# Autodesk Inventor assembly: ASY GBK 3330 central wall shield 9
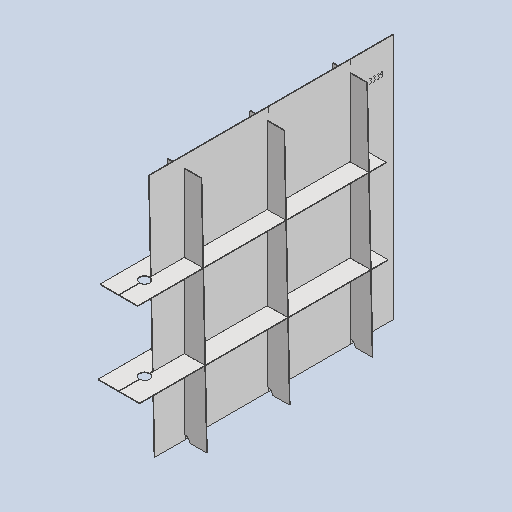
[picture p0: Inventor's stored thumbnail of the model, 512x512]
Saved by Autodesk Inventor 2026.3 (Build 303398000, 398)
## iProperties
Created: 2026-05-19
Part Number: ASY GBK 3330 central wall shield 9
Document SubType Name: Assembly
Designer: pokla
Mass: 123029 g
Surface Area: 79995.2 cm^2
Volume: 15672.5 cm^3
Density: 7.85 g/cm^3
Stock Number: 3330
Author: admin
## Documents named in this file (7)
- C:\Users\admin\Documents\Inventor\GBK-Gubkinskiy\ASY GBK 3330 central wall shield 9.iam
- C:\Users\admin\Documents\Inventor\GBK-Gubkinskiy\GBK 0101 main rib.ipt
- C:\Users\admin\Documents\Inventor\GBK-Gubkinskiy\GBK 3339 shield 9.ipt
- C:\Users\admin\Documents\Inventor\GBK-Gubkinskiy\GBK 3311 central third rib_CPY1.ipt
- GBK 3311 central third rib_CPY1.ipt
- C:\Users\admin\Documents\Inventor\GBK-Gubkinskiy\GBK 3312 stringer 7.ipt
- C:\Users\admin\Documents\Inventor\GBK-Gubkinskiy\GBK 3313 stringer 8.ipt
## Components (11 placed, 4 different names)
1. GBK 3312 stringer 7:1 — Rigid:1
2. GBK 3339 shield 9:1 — Mate:1, Mate:2, Mate:4, Flush:6, Mate:5, Flush:7, Flush:6
3. GBK 3313 stringer 8:1 — Rigid:2, Rigid:7, Rigid:8
4. GBK 3312 stringer 7:2 — Rigid:4
5. GBK 3313 stringer 8:2 — Rigid:3, Flush:6, Rigid:5, Rigid:6
6. GBK 3311 central third rib_CPY1:2 — Flush:4, Mate:5, Flush:7, Rigid:2, Rigid:1
7. GBK 3311 central third rib_CPY1:1 — Mate:4, Flush:6, Flush:4, Rigid:3, Rigid:4
8. GBK 3311 central third rib_CPY1:3 — Rigid:5
9. GBK 3311 central third rib_CPY1:4 — Rigid:6
10. GBK 3311 central third rib_CPY1:5 — Rigid:7
11. GBK 3311 central third rib_CPY1:6 — Rigid:8
## Relationships (16: WeldJoint 8, Mate 4, Flush 4)
- Mate:1: GBK 3339 shield 9:1
- Mate:2: GBK 3339 shield 9:1
- Mate:4: GBK 3339 shield 9:1 ↔ GBK 3311 central third rib_CPY1:1
- Flush:6: GBK 3339 shield 9:1 ↔ GBK 3311 central third rib_CPY1:1
- Flush:4: GBK 3311 central third rib_CPY1:2 ↔ GBK 3311 central third rib_CPY1:1
- Mate:5: GBK 3339 shield 9:1 ↔ GBK 3311 central third rib_CPY1:2
- Flush:7: GBK 3339 shield 9:1 ↔ GBK 3311 central third rib_CPY1:2
- Rigid:3 [WeldJoint] (4 mm): GBK 3313 stringer 8:2 ↔ GBK 3311 central third rib_CPY1:1
- Rigid:4 [WeldJoint] (4 mm): GBK 3312 stringer 7:2 ↔ GBK 3311 central third rib_CPY1:1
- Rigid:2 [WeldJoint] (4 mm): GBK 3313 stringer 8:1 ↔ GBK 3311 central third rib_CPY1:2
- Rigid:1 [WeldJoint] (4 mm): GBK 3312 stringer 7:1 ↔ GBK 3311 central third rib_CPY1:2
- Flush:6 (155 mm): GBK 3339 shield 9:1 ↔ GBK 3313 stringer 8:2
- Rigid:5 [WeldJoint] (4 mm): GBK 3313 stringer 8:2 ↔ GBK 3311 central third rib_CPY1:3
- Rigid:6 [WeldJoint] (4 mm): GBK 3313 stringer 8:2 ↔ GBK 3311 central third rib_CPY1:4
- Rigid:7 [WeldJoint] (4 mm): GBK 3313 stringer 8:1 ↔ GBK 3311 central third rib_CPY1:5
- Rigid:8 [WeldJoint] (4 mm): GBK 3313 stringer 8:1 ↔ GBK 3311 central third rib_CPY1:6
## Named parameters: основание_длина_нижнего = 200 mm, основание_длина_верхнего = 100 mm, стрингер_глубина_1 = 190.70056 mm, стрингер_глубина_2 = 179.35977 mm, стрингер_глубина_3 = 168.01899 mm, стрингер_глубина_4 = 156.6782 mm, стрингер_глубина_5 = 145.33742 mm, стрингер_глубина_6 = 133.99663 mm, стрингер_глубина_7 = 122.65585 mm, стрингер_глубина_8 = 111.31507 mm, Лист_ширина = 1480 mm, ребро_усилителей = 60 mm, паз_под_стрингер_глубина = 70 mm, паз_под_стрингер_толщина = 5 mm, отступ_от_пола_до_первого_стрингера = 410 mm, шаг_стрингеров = 500 mm, радиус_выреза_под_сварку = 30 mm, нахлест_шпангоутов_1_2 = 150 mm, нахлест_шпангоутов_2_3 = 120 mm, Стрингер_длина = 1489.5 mm, Лист_длина = 2980 mm, Шаг_шпангоутов = 496.66667 mm
